# Autodesk Inventor assembly: a
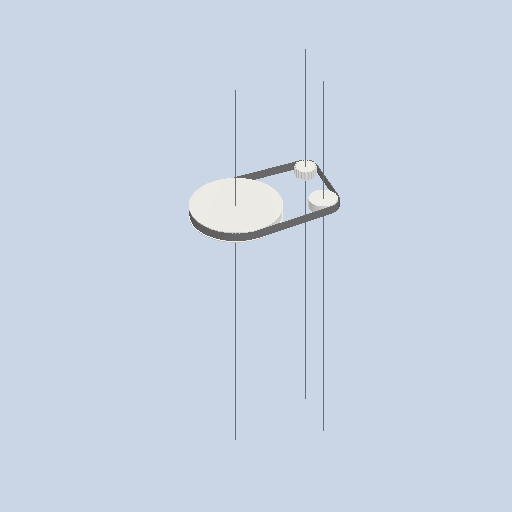
[picture p0: Inventor's stored thumbnail of the model, 512x512]
Saved by Autodesk Inventor 2024 (Build 280153000, 153)
## iProperties
ClientObjectVersion: 1
Created: 2023-11-23
Part Number: a
Document SubType Name: Assembly
Designer: mb
Author: mb
Title: a
Subject: a
## Documents named in this file (5)
- C:\Users\MaartenGeorgesBuelen\Documents\Inventor\robot arm\base\Design Accelerator\Synchronous Belts Transmission2.iam
- C:\Users\MaartenGeorgesBuelen\Documents\Inventor\robot arm\base\Design Accelerator\Synchronous Belt2.ipt
- C:\Users\MaartenGeorgesBuelen\Documents\Inventor\robot arm\base\Design Accelerator\Synchronous Pulley12.ipt
- C:\Users\MaartenGeorgesBuelen\Documents\Inventor\robot arm\base\Design Accelerator\Synchronous Pulley22.ipt
- C:\Users\MaartenGeorgesBuelen\Documents\Inventor\robot arm\base\Design Accelerator\Flat Pulley11.ipt
## Components (4 placed, 4 different names)
1. Synchronous Belt:1 — Flush:1, Mate:1, Mate:2, Flush:2, Mate:3, Mate:4, Flush:3, Mate:5
2. Synchronous Pulley1:1 — Flush:1, Mate:1, Mate:2, Rotation:1, Rotation:2
3. Synchronous Pulley2:1 — Flush:2, Mate:3, Rotation:1, Mate:4
4. Flat Pulley1:1 — Flush:3, Mate:5, Rotation:2
## Relationships (10: Mate 5, Flush 3, RelateRotation 2)
- Flush:1: Synchronous Belt:1 ↔ Synchronous Pulley1:1
- Mate:1: Synchronous Belt:1 ↔ Synchronous Pulley1:1
- Mate:2: Synchronous Belt:1 ↔ Synchronous Pulley1:1
- Flush:2: Synchronous Belt:1 ↔ Synchronous Pulley2:1
- Mate:3: Synchronous Belt:1 ↔ Synchronous Pulley2:1
- Rotation:1 [RelateRotation] (4 ul): Synchronous Pulley1:1 ↔ Synchronous Pulley2:1
- Mate:4: Synchronous Belt:1 ↔ Synchronous Pulley2:1
- Flush:3: Synchronous Belt:1 ↔ Flat Pulley1:1
- Mate:5: Synchronous Belt:1 ↔ Flat Pulley1:1
- Rotation:2 [RelateRotation] (1.3823 ul): Synchronous Pulley1:1 ↔ Flat Pulley1:1
